# Autodesk Inventor assembly: RT_ARM_A_001
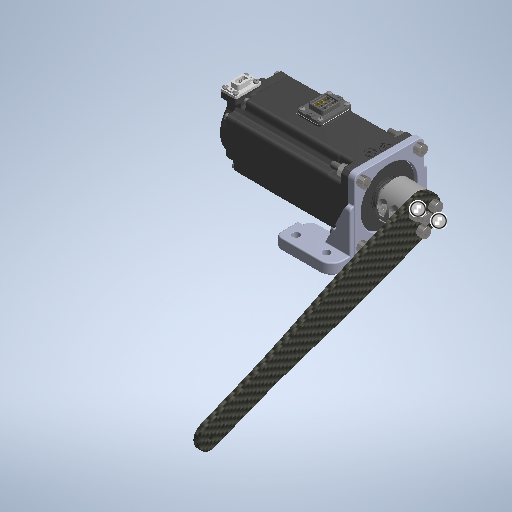
[picture p0: Inventor's stored thumbnail of the model, 512x512]
Saved by Autodesk Inventor 2025.3 (Build 293356000, 356)
## iProperties
Part Number: RT_ARM_A_001
Document SubType Name: Assembly
Designer: louis
Author: louis
## Documents named in this file (9)
- C:\Users\louis\OneDrive\Desktop\R_Trident\02_CAD\04_Subassemblies\RT_ARM_A_001.iam
- C:\Users\louis\OneDrive\Desktop\R_Trident\02_CAD\03_Parts_Custom\RT_ARM_MC_002.ipt
- C:\Users\louis\OneDrive\Desktop\R_Trident\02_CAD\01_Standard_Parts\A6M60-400H2B1-M17\A6M60-400H2B1-M17.iam
- C:\Users\louis\OneDrive\Desktop\R_Trident\02_CAD\01_Standard_Parts\ST-M4\ST-M4.ipt
- C:\Users\louis\OneDrive\Documents\Inventor\Content Center Files\R2025\en-US\ISO 4762(2)\ISO 4762 - M5 x 25ISO.ipt
- C:\Users\louis\OneDrive\Documents\Inventor\Content Center Files\R2025\en-US\ISO 4032(2)\ISO 4032 - M5 - ISO.ipt
- C:\Users\louis\OneDrive\Desktop\R_Trident\02_CAD\03_Parts_Custom\RT_DRV_MC_003_ShaftCoupling.ipt
- C:\Users\louis\OneDrive\Documents\Inventor\Content Center Files\R2025\en-US\ISO 4762(2)\ISO 4762 - M5 x 8ISO.ipt
- C:\Users\louis\OneDrive\Documents\Inventor\Content Center Files\R2025\en-US\ISO 4762(2)\ISO 4762 - M4 x 6ISO.ipt
## Components (18 placed, 8 different names)
1. ISO 4762 M4 x 6:2 — Mate:33, Mate:34
2. ISO 4762 M4 x 6:1 — Mate:31, Mate:32
3. ISO 4762 M5 x 8:3 — Mate:29, Mate:30
4. ISO 4762 M5 x 8:2 — Mate:27, Mate:28
5. ISO 4762 M5 x 8:1 — Mate:25, Mate:26
6. RT_DRV_MC_003_ShaftCoupling:1 — Mate:20, Mate:21, Flush:2, Mate:23, Mate:24, Mate:25, Mate:27, Mate:29, Mate:31, Mate:32, Mate:33, Mate:34
7. ISO 4762 M5 x 25:6 — Insert:10, Mate:22
8. RT_ARM_MC_002:1 — Insert:10, Mate:23, Mate:24, Mate:26, Mate:28, Mate:30
9. A6M60-400H2B1-M17:1 [sub-assembly] — Mate:15, Mate:16, Mate:17, Insert:5, Insert:6, Insert:7, Insert:8, Flush:1, Mate:19, Mate:20, Mate:21, Flush:2, Mate:22
10. ST-M4:1 — Mate:15, Mate:16, Mate:17, Mate:18, Insert:1, Insert:2, Insert:3, Insert:4
11. ISO 4762 M5 x 25:1 — Insert:1
12. ISO 4762 M5 x 25:2 — Insert:2
13. ISO 4762 M5 x 25:3 — Insert:3
14. ISO 4762 M5 x 25:4 — Insert:4
15. ISO 4032 M5:1 — Insert:5
16. ISO 4032 M5:2 — Insert:6
17. ISO 4032 M5:3 — Insert:7
18. ISO 4032 M5:4 — Insert:8
## Relationships (31: Mate 20, Insert 9, Flush 2)
- Mate:15: A6M60-400H2B1-M17:1 ↔ ST-M4:1
- Mate:16: A6M60-400H2B1-M17:1 ↔ ST-M4:1
- Mate:17: A6M60-400H2B1-M17:1 ↔ ST-M4:1
- Mate:18: ST-M4:1
- Insert:1: ST-M4:1 ↔ ISO 4762 M5 x 25:1
- Insert:2: ST-M4:1 ↔ ISO 4762 M5 x 25:2
- Insert:3: ST-M4:1 ↔ ISO 4762 M5 x 25:3
- Insert:4: ST-M4:1 ↔ ISO 4762 M5 x 25:4
- Insert:5: A6M60-400H2B1-M17:1 ↔ ISO 4032 M5:1
- Insert:6: A6M60-400H2B1-M17:1 ↔ ISO 4032 M5:2
- Insert:7: A6M60-400H2B1-M17:1 ↔ ISO 4032 M5:3
- Insert:8: A6M60-400H2B1-M17:1 ↔ ISO 4032 M5:4
- Flush:1: A6M60-400H2B1-M17:1
- Mate:19: A6M60-400H2B1-M17:1
- Insert:10: ISO 4762 M5 x 25:6 ↔ RT_ARM_MC_002:1
- Mate:20: RT_DRV_MC_003_ShaftCoupling:1 ↔ A6M60-400H2B1-M17:1
- Mate:21: RT_DRV_MC_003_ShaftCoupling:1 ↔ A6M60-400H2B1-M17:1
- Flush:2: RT_DRV_MC_003_ShaftCoupling:1 ↔ A6M60-400H2B1-M17:1
- Mate:22: ISO 4762 M5 x 25:6 ↔ A6M60-400H2B1-M17:1
- Mate:23: RT_DRV_MC_003_ShaftCoupling:1 ↔ RT_ARM_MC_002:1
- Mate:24: RT_DRV_MC_003_ShaftCoupling:1 ↔ RT_ARM_MC_002:1
- Mate:25: ISO 4762 M5 x 8:1 ↔ RT_DRV_MC_003_ShaftCoupling:1
- Mate:26: ISO 4762 M5 x 8:1 ↔ RT_ARM_MC_002:1
- Mate:27: ISO 4762 M5 x 8:2 ↔ RT_DRV_MC_003_ShaftCoupling:1
- Mate:28: ISO 4762 M5 x 8:2 ↔ RT_ARM_MC_002:1
- Mate:29: ISO 4762 M5 x 8:3 ↔ RT_DRV_MC_003_ShaftCoupling:1
- Mate:30: ISO 4762 M5 x 8:3 ↔ RT_ARM_MC_002:1
- Mate:31: ISO 4762 M4 x 6:1 ↔ RT_DRV_MC_003_ShaftCoupling:1
- Mate:32: ISO 4762 M4 x 6:1 ↔ RT_DRV_MC_003_ShaftCoupling:1
- Mate:33: ISO 4762 M4 x 6:2 ↔ RT_DRV_MC_003_ShaftCoupling:1
- Mate:34: ISO 4762 M4 x 6:2 ↔ RT_DRV_MC_003_ShaftCoupling:1
